# Autodesk Inventor assembly: cajas
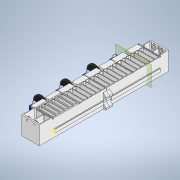
[picture p0: Inventor's stored thumbnail of the model, 180x180]
Saved by Autodesk Inventor 2020.3 (Build 243373000, 373)
## iProperties
Created: 2021-02-18
Part Number: cajas
Document SubType Name: Assembly
Designer: juanp
Author: juanp
## Documents named in this file (7)
- C:\Users\juanp\Desktop\Robocol\Nuevo EVA\V1\Cajas\cajas.iam
- C:\Users\juanp\Desktop\Robocol\Nuevo EVA\V1\Cajas\Solid1_1.ipt
- C:\Users\juanp\Desktop\Robocol\Nuevo EVA\V1\Cajas\Puerta Cremallera.ipt
- C:\Users\juanp\Desktop\Robocol\Nuevo EVA\V1\Cajas\Engranaje.ipt
- C:\Users\juanp\Desktop\Robocol\Nuevo EVA\Recursos\Servo SG90\SG90 - Micro Servo 9g - Tower Pro.iam
- C:\Users\juanp\Desktop\Robocol\Nuevo EVA\V1\Cajas\Adaptador SG90.ipt
- C:\Users\juanp\Desktop\Robocol\Nuevo EVA\V1\Cajas\Solid11.ipt
## Components (18 placed, 6 different names)
1. Solid1_1:1 — Mate:2, Mate:3, Mate:5, Angle:1, Mate:13, Mate:14, Mate:16, Mate:18, Mate:19, Mate:20, Mate:36, Mate:37, Mate:38, Mate:39, Mate:40, Mate:41, Mate:42, Mate:43, Mate:44
2. Puerta Cremallera:1 — Mate:2, Mate:3, Mate:4, Mate:9, Rotation/Translation:1, Flush:1
3. Engranaje:1 — Mate:4, Mate:5, Mate:7, Mate:8, Mate:9, Rotation/Translation:1, Mate:47
4. SG90 - Micro Servo 9g - Tower Pro:1 [sub-assembly] — Mate:7, Mate:8, Angle:1, Mate:11, Mate:12
5. Adaptador SG90:1 — Mate:11, Mate:12
6. Puerta Cremallera:2 — Mate:13, Mate:14, Flush:1, Flush:2
7. Puerta Cremallera:3 — Mate:19, Mate:20, Flush:2, Flush:3
8. Puerta Cremallera:4 — Mate:16, Mate:18, Flush:3
9. Engranaje:2 — Mate:45, Mate:47
10. SG90 - Micro Servo 9g - Tower Pro:2 [sub-assembly] — Mate:49
11. Adaptador SG90:2 — Mate:39, Mate:40, Mate:41, Mate:49
12. Engranaje:3 — Mate:45, Mate:46
13. SG90 - Micro Servo 9g - Tower Pro:3 [sub-assembly] — Mate:50
14. Adaptador SG90:3 — Mate:42, Mate:43, Mate:44, Mate:50
15. Engranaje:4 — Mate:46
16. SG90 - Micro Servo 9g - Tower Pro:4 [sub-assembly] — Mate:48
17. Adaptador SG90:4 — Mate:36, Mate:37, Mate:38, Mate:48
18. Solid11:1
## Relationships (47: Mate 42, Flush 3, RelateRotateTranslate 1, Angle 1)
- Mate:2: Solid1_1:1 ↔ Puerta Cremallera:1
- Mate:3: Solid1_1:1 ↔ Puerta Cremallera:1
- Mate:4: Puerta Cremallera:1 ↔ Engranaje:1
- Mate:5 (25 mm): Solid1_1:1 ↔ Engranaje:1
- Mate:7: Engranaje:1 ↔ SG90 - Micro Servo 9g - Tower Pro:1
- Mate:8: Engranaje:1 ↔ SG90 - Micro Servo 9g - Tower Pro:1
- Mate:9 (20 mm): Puerta Cremallera:1 ↔ Engranaje:1
- Rotation/Translation:1 [RelateRotateTranslate] (125.6637 mm): Puerta Cremallera:1 ↔ Engranaje:1
- Angle:1 (90 deg): Solid1_1:1 ↔ SG90 - Micro Servo 9g - Tower Pro:1
- Mate:11: SG90 - Micro Servo 9g - Tower Pro:1 ↔ Adaptador SG90:1
- Mate:12: SG90 - Micro Servo 9g - Tower Pro:1 ↔ Adaptador SG90:1
- Mate:13: Solid1_1:1 ↔ Puerta Cremallera:2
- Mate:14: Solid1_1:1 ↔ Puerta Cremallera:2
- Mate:16: Solid1_1:1 ↔ Puerta Cremallera:4
- Mate:18: Solid1_1:1 ↔ Puerta Cremallera:4
- Mate:19: Solid1_1:1 ↔ Puerta Cremallera:3
- Mate:20: Solid1_1:1 ↔ Puerta Cremallera:3
- [Mate]: Engranaje:2 ↔ SG90 - Micro Servo 9g - Tower Pro:2
- [Mate]: Engranaje:2 ↔ SG90 - Micro Servo 9g - Tower Pro:2
- [Mate]: SG90 - Micro Servo 9g - Tower Pro:2 ↔ Adaptador SG90:2
- [Mate]: SG90 - Micro Servo 9g - Tower Pro:2 ↔ Adaptador SG90:2
- [Mate]: Engranaje:3 ↔ SG90 - Micro Servo 9g - Tower Pro:3
- [Mate]: Engranaje:3 ↔ SG90 - Micro Servo 9g - Tower Pro:3
- [Mate]: SG90 - Micro Servo 9g - Tower Pro:3 ↔ Adaptador SG90:3
- [Mate]: SG90 - Micro Servo 9g - Tower Pro:3 ↔ Adaptador SG90:3
- [Mate]: Engranaje:4 ↔ SG90 - Micro Servo 9g - Tower Pro:4
- [Mate]: Engranaje:4 ↔ SG90 - Micro Servo 9g - Tower Pro:4
- [Mate]: SG90 - Micro Servo 9g - Tower Pro:4 ↔ Adaptador SG90:4
- [Mate]: SG90 - Micro Servo 9g - Tower Pro:4 ↔ Adaptador SG90:4
- Mate:36: Solid1_1:1 ↔ Adaptador SG90:4
- Mate:37: Solid1_1:1 ↔ Adaptador SG90:4
- Mate:38: Solid1_1:1 ↔ Adaptador SG90:4
- Mate:39: Solid1_1:1 ↔ Adaptador SG90:2
- Mate:40: Solid1_1:1 ↔ Adaptador SG90:2
- Mate:41: Solid1_1:1 ↔ Adaptador SG90:2
- Mate:42: Solid1_1:1 ↔ Adaptador SG90:3
- Mate:43: Solid1_1:1 ↔ Adaptador SG90:3
- Mate:44: Solid1_1:1 ↔ Adaptador SG90:3
- Flush:1: Puerta Cremallera:1 ↔ Puerta Cremallera:2
- Flush:2: Puerta Cremallera:2 ↔ Puerta Cremallera:3
- Flush:3: Puerta Cremallera:3 ↔ Puerta Cremallera:4
- Mate:45: Engranaje:2 ↔ Engranaje:3
- Mate:46: Engranaje:3 ↔ Engranaje:4
- Mate:47: Engranaje:1 ↔ Engranaje:2
- Mate:48: SG90 - Micro Servo 9g - Tower Pro:4 ↔ Adaptador SG90:4
- Mate:49: SG90 - Micro Servo 9g - Tower Pro:2 ↔ Adaptador SG90:2
- Mate:50: SG90 - Micro Servo 9g - Tower Pro:3 ↔ Adaptador SG90:3
## Named parameters: d35_d14 = 0 mm, d36_d15 = 0 mm, d38_d24 = 0 mm, d39_d25 = 0 mm, d40_d14 = 0 mm, d41_d15 = 0 mm, d43_d24 = 0 mm, d44_d25 = 0 mm, d45_d14 = 0 mm, d46_d15 = 0 mm, d48_d24 = 0 mm, d49_d25 = 0 mm
